# Autodesk Inventor assembly: camera-lens-mount-assembly
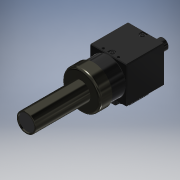
[picture p0: Inventor's stored thumbnail of the model, 180x180]
Saved by Autodesk Inventor 2019 (Build 230136000, 136)
## iProperties
Created: 2019-03-10
Part Number: camera-lens-mount-assembly
Document SubType Name: Assembly
Designer: Wilson Lab
Author: Wilson Lab
## Documents named in this file (4)
- C:\code\auditory-behavior-experiments\design-files\camera-assembly\camera-lens-mount-assembly.iam
- C:\code\auditory-behavior-experiments\design-files\camera-assembly\FL2-020-R0.ipt
- C:\code\auditory-behavior-experiments\design-files\camera-assembly\Flea2 Tripod Adapter.ipt
- C:\code\auditory-behavior-experiments\design-files\camera-assembly\InfiniStix_066x.ipt
## Components (3 placed, 3 different names)
1. FL2-020-R0:1 — Rigid:1, Rigid:2
2. Flea2 Tripod Adapter:1 — Rigid:2
3. InfiniStix_066x:1 — Rigid:1
## Relationships (2: WeldJoint 2)
- Rigid:1 [WeldJoint]: FL2-020-R0:1 ↔ InfiniStix_066x:1
- Rigid:2 [WeldJoint]: FL2-020-R0:1 ↔ Flea2 Tripod Adapter:1
